# Autodesk Inventor assembly: AK-C-C39-vertival
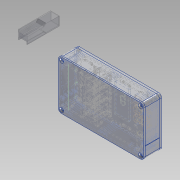
[picture p0: Inventor's stored thumbnail of the model, 180x180]
Saved by Autodesk Inventor 2016 (Build 200138000, 138)
## iProperties
Created: 2016-04-02
Part Number: AK-C-C39-vertival
Document SubType Name: Assembly
Designer: admin
Author: admin
## Documents named in this file (15)
- E:\Alex\DI-Lambda\parts\v1\AK-C-C39\AK-C-C39-DI-Lambda-v1.iam
- E:\Alex\DI-Lambda\parts\Common\SZOMK-AK-C-C39.ipt
- E:\Alex\DI-Lambda\parts\v1\AK-C-C39\AK-C-C39-Top.ipt
- E:\Alex\DI-Lambda\parts\v1\AK-C-C39\AK-C-C39-Main-Board.ipt
- E:\Alex\DI-Lambda\parts\v1\AK-C-C39\AK-C-C39-Separator.ipt
- E:\Alex\DI-Lambda\parts\v1\AK-C-C39\AK-C-C39-Pinhole-Board.ipt
- E:\Alex\DI-Lambda\parts\v1\AK-C-C39\AK-C-C39-LED-Board-Assembly.iam
- E:\Alex\DI-Lambda\parts\v1\AK-C-C39\AK-C-C39-Sensor-Board.ipt
- E:\Alex\DI-Lambda\parts\v1\AK-C-C39\AK-C-C39-Bottom.ipt
- E:\Alex\DI-Lambda\parts\Common\Cuvette.ipt
- E:\Alex\DI-Lambda\parts\Common\Paper-holder.iam
- E:\Alex\DI-Lambda\parts\v1\AK-C-C39\LCD.ipt
- E:\Alex\DI-Lambda\parts\Common\Button.ipt
- C:\Users\admin\Documents\Inventor\Content Center Files\R2016\en-US\SS-ISO 7046  Z\ISO 7046-1 - M3 x 8Z.ipt
- E:\Alex\DI-Lambda\parts\v1\AK-C-C39\AK-C-C39-Holder-IM.ipt
## Components (24 placed, 14 different names)
1. SZOMK-AK-C-C39:1 — Mate:1, Mate:2, Mate:3, Mate:36, Mate:37, Mate:38
2. AK-C-C39-Top:1 — Mate:1, Mate:2, Mate:3, Mate:4, Mate:48, Mate:49, Mate:68, Mate:69, Mate:70, Mate:71, Flush:1, Flush:2, Flush:3, Flush:4, Mate:72, Mate:73, Mate:74, Mate:75, Mate:76, Mate:77, Mate:78, Mate:79, Mate:80, Mate:81, Mate:82, Mate:83, Mate:86, Mate:87, Mate:98, Mate:99
3. AK-C-C39-Main-Board:1 — Mate:4, Mate:25, Mate:29, Mate:30, Mate:32, Mate:33, Mate:35, Mate:47, Mate:50, Mate:51, Mate:52, Mate:53, Mate:54, Mate:55, Mate:84, Mate:85, Mate:86, Mate:87, Mate:88, Mate:89, Mate:90, Mate:91, Mate:92, Mate:93, Mate:94, Mate:95, Mate:96, Mate:97, Mate:100
4. AK-C-C39-Separator:1 — Mate:25, Mate:85, Mate:94
5. AK-C-C39-Separator:2 — Mate:35, Mate:84, Mate:95
6. AK-C-C39-LED-Board-Assembly:1 [sub-assembly] — Mate:32, Mate:33, Mate:96
7. AK-C-C39-Sensor-Board:1 — Mate:29, Mate:30, Mate:100
8. AK-C-C39-Bottom:1 — Mate:36, Mate:37, Mate:38, Mate:46
9. Cuvette:1
10. Paper-holder:1 [sub-assembly] — Mate:46
11. LCD:1 — Mate:47, Mate:48, Mate:49
12. Button:1 — Mate:50, Mate:82, Mate:83
13. Button:2 — Mate:51, Mate:78, Mate:79
14. Button:3 — Mate:52, Mate:72, Mate:73
15. Button:4 — Mate:53, Mate:80, Mate:81
16. Button:5 — Mate:54, Mate:76, Mate:77
17. Button:6 — Mate:55, Mate:74, Mate:75
18. SS ISO 7046 Z M3 x 8:1 — Mate:68, Flush:1
19. SS ISO 7046 Z M3 x 8:2 — Mate:69, Flush:2
20. SS ISO 7046 Z M3 x 8:3 — Mate:70, Flush:3
21. SS ISO 7046 Z M3 x 8:4 — Mate:71, Flush:4
22. AK-C-C39-Pinhole-Board:1 — Mate:88, Mate:90, Mate:91
23. AK-C-C39-Pinhole-Board:2 — Mate:89, Mate:92, Mate:93
24. AK-C-C39-Holder-IM:1 — Mate:97, Mate:98, Mate:99
## Relationships (60: Mate 56, Flush 4)
- Mate:1: SZOMK-AK-C-C39:1 ↔ AK-C-C39-Top:1
- Mate:2: SZOMK-AK-C-C39:1 ↔ AK-C-C39-Top:1
- Mate:3: SZOMK-AK-C-C39:1 ↔ AK-C-C39-Top:1
- Mate:4: AK-C-C39-Top:1 ↔ AK-C-C39-Main-Board:1
- Mate:25: AK-C-C39-Main-Board:1 ↔ AK-C-C39-Separator:1
- Mate:29: AK-C-C39-Main-Board:1 ↔ AK-C-C39-Sensor-Board:1
- Mate:30: AK-C-C39-Main-Board:1 ↔ AK-C-C39-Sensor-Board:1
- Mate:32: AK-C-C39-Main-Board:1 ↔ AK-C-C39-LED-Board-Assembly:1
- Mate:33: AK-C-C39-Main-Board:1 ↔ AK-C-C39-LED-Board-Assembly:1
- Mate:35: AK-C-C39-Main-Board:1 ↔ AK-C-C39-Separator:2
- Mate:36: SZOMK-AK-C-C39:1 ↔ AK-C-C39-Bottom:1
- Mate:37: SZOMK-AK-C-C39:1 ↔ AK-C-C39-Bottom:1
- Mate:38: SZOMK-AK-C-C39:1 ↔ AK-C-C39-Bottom:1
- Mate:46: AK-C-C39-Bottom:1 ↔ Paper-holder:1
- Mate:47: AK-C-C39-Main-Board:1 ↔ LCD:1
- Mate:48: AK-C-C39-Top:1 ↔ LCD:1
- Mate:49: AK-C-C39-Top:1 ↔ LCD:1
- Mate:50: AK-C-C39-Main-Board:1 ↔ Button:1
- Mate:51: AK-C-C39-Main-Board:1 ↔ Button:2
- Mate:52: AK-C-C39-Main-Board:1 ↔ Button:3
- Mate:53: AK-C-C39-Main-Board:1 ↔ Button:4
- Mate:54: AK-C-C39-Main-Board:1 ↔ Button:5
- Mate:55: AK-C-C39-Main-Board:1 ↔ Button:6
- Mate:68: AK-C-C39-Top:1 ↔ SS ISO 7046 Z M3 x 8:1
- Mate:69: AK-C-C39-Top:1 ↔ SS ISO 7046 Z M3 x 8:2
- Mate:70: AK-C-C39-Top:1 ↔ SS ISO 7046 Z M3 x 8:3
- Mate:71: AK-C-C39-Top:1 ↔ SS ISO 7046 Z M3 x 8:4
- Flush:1: AK-C-C39-Top:1 ↔ SS ISO 7046 Z M3 x 8:1
- Flush:2: AK-C-C39-Top:1 ↔ SS ISO 7046 Z M3 x 8:2
- Flush:3: AK-C-C39-Top:1 ↔ SS ISO 7046 Z M3 x 8:3
- Flush:4: AK-C-C39-Top:1 ↔ SS ISO 7046 Z M3 x 8:4
- Mate:72: AK-C-C39-Top:1 ↔ Button:3
- Mate:73: AK-C-C39-Top:1 ↔ Button:3
- Mate:74: AK-C-C39-Top:1 ↔ Button:6
- Mate:75: AK-C-C39-Top:1 ↔ Button:6
- Mate:76: AK-C-C39-Top:1 ↔ Button:5
- Mate:77: AK-C-C39-Top:1 ↔ Button:5
- Mate:78: AK-C-C39-Top:1 ↔ Button:2
- Mate:79: AK-C-C39-Top:1 ↔ Button:2
- Mate:80: AK-C-C39-Top:1 ↔ Button:4
- Mate:81: AK-C-C39-Top:1 ↔ Button:4
- Mate:82: AK-C-C39-Top:1 ↔ Button:1
- Mate:83: AK-C-C39-Top:1 ↔ Button:1
- Mate:84: AK-C-C39-Main-Board:1 ↔ AK-C-C39-Separator:2
- Mate:85: AK-C-C39-Main-Board:1 ↔ AK-C-C39-Separator:1
- Mate:86: AK-C-C39-Top:1 ↔ AK-C-C39-Main-Board:1
- Mate:87: AK-C-C39-Top:1 ↔ AK-C-C39-Main-Board:1
- Mate:88: AK-C-C39-Main-Board:1 ↔ AK-C-C39-Pinhole-Board:1
- Mate:89: AK-C-C39-Main-Board:1 ↔ AK-C-C39-Pinhole-Board:2
- Mate:90: AK-C-C39-Main-Board:1 ↔ AK-C-C39-Pinhole-Board:1
- Mate:91: AK-C-C39-Main-Board:1 ↔ AK-C-C39-Pinhole-Board:1
- Mate:92: AK-C-C39-Main-Board:1 ↔ AK-C-C39-Pinhole-Board:2
- Mate:93: AK-C-C39-Main-Board:1 ↔ AK-C-C39-Pinhole-Board:2
- Mate:94: AK-C-C39-Main-Board:1 ↔ AK-C-C39-Separator:1
- Mate:95: AK-C-C39-Main-Board:1 ↔ AK-C-C39-Separator:2
- Mate:96: AK-C-C39-Main-Board:1 ↔ AK-C-C39-LED-Board-Assembly:1
- Mate:97: AK-C-C39-Main-Board:1 ↔ AK-C-C39-Holder-IM:1
- Mate:98: AK-C-C39-Top:1 ↔ AK-C-C39-Holder-IM:1
- Mate:99: AK-C-C39-Top:1 ↔ AK-C-C39-Holder-IM:1
- Mate:100: AK-C-C39-Main-Board:1 ↔ AK-C-C39-Sensor-Board:1
